# Autodesk Inventor assembly: ElevatorCar
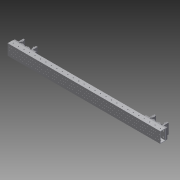
[picture p0: Inventor's stored thumbnail of the model, 180x180]
Saved by Autodesk Inventor 2015 (Build 190159000, 159)
## iProperties
Created: 2015-01-25
Part Number: ElevatorCar
Document SubType Name: Assembly
Designer: cstewart1
Author: cstewart1
## Documents named in this file (3)
- C:\Users\cstewart1\Inventor\HWRobot2015CAD\Elevator\ElevatorCar.iam
- C:\Users\cstewart1\Inventor\HWRobot2015CAD\FRCKOP2015\McMaster\60585K370.ipt
- C:\Users\cstewart1\Inventor\HWRobot2015CAD\FRCKOP2015\VersaFrame\217-3453-STEP.ipt
## Components (3 placed, 3 different names)
1. LeftTrolly — Mate:1, Flush:1, Flush:2, Mate:3
2. CrossBar — Mate:1, Flush:1, Flush:2, Mate:2, Flush:3
3. RightTrolly — Mate:2, Flush:3, Mate:3
## Relationships (6: Mate 3, Flush 3)
- Mate:1: LeftTrolly ↔ CrossBar
- Flush:1: LeftTrolly ↔ CrossBar
- Flush:2 (-1.524 mm): LeftTrolly ↔ CrossBar
- Mate:2: CrossBar ↔ RightTrolly
- Flush:3 (1.524 mm): CrossBar ↔ RightTrolly
- Mate:3 (509.651 mm): LeftTrolly ↔ RightTrolly
